# Autodesk Inventor assembly: Leg_joint_roll_yaw
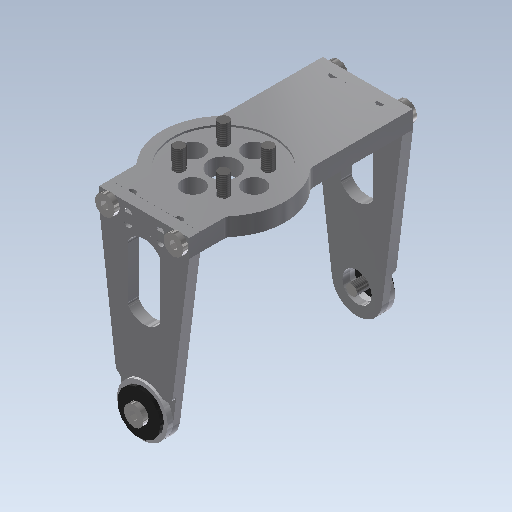
[picture p0: Inventor's stored thumbnail of the model, 512x512]
Saved by Autodesk Inventor 2020 (Build 240168000, 168)
## iProperties
Created: 2016-05-01
Part Number: Leg_joint_roll_yaw
Document SubType Name: Assembly
Designer: hiroaki
Mass: 101.489 g
Surface Area: 218.083 cm^2
Volume: 17.9148 cm^3
Density: 5.6651 g/cm^3
Author: hiroaki
## Documents named in this file (7)
- C:\Users\Masato\Documents\Inventor\CIT Brains_Inventor\OpenPlatform_ver3_0\LowerBody\Leg_joit\Leg_joint_roll_yaw.iam
- C:\Users\Masato\Documents\Inventor\CIT Brains_Inventor\OpenPlatform_ver3_0\Ready_Made\UUW-0312-10BH.ipt
- C:\Users\Masato\Documents\Inventor\CIT Brains_Inventor\OpenPlatform_ver3_0\LowerBody\Leg_joit\Leg_joint_yaw_frame.ipt
- C:\Users\Masato\Documents\Inventor\CIT Brains_Inventor\OpenPlatform_ver3_0\Ready_Made\Screw\M3-10.ipt
- C:\Users\Masato\Documents\Inventor\CIT Brains_Inventor\OpenPlatform_ver3_0\Ready_Made\Screw\M3-6.ipt
- C:\Users\Masato\Documents\Inventor\CIT Brains_Inventor\OpenPlatform_ver3_0\Ready_Made\TT-0814-15.ipt
- C:\Users\Masato\Documents\Inventor\CIT Brains_Inventor\OpenPlatform_ver3_0\LowerBody\Leg_joit\Leg_joint_slider_frame.ipt
## Components (17 placed, 6 different names)
1. UUW-0312-10BH:3 — 挿入:63, 挿入:76
2. UUW-0312-10BH:4 — 挿入:64, 挿入:77
3. Leg_joint_yaw_frame:1 — 挿入:53, 挿入:54, 挿入:55, 挿入:56, 挿入:66, 挿入:67, 挿入:71, 挿入:72
4. M3-10:1 — 挿入:53
5. M3-10:2 — 挿入:54
6. M3-10:3 — 挿入:55
7. M3-10:4 — 挿入:56
8. M3-6:1 — 挿入:74
9. M3-6:2 — 挿入:73
10. M3-6:3 — 挿入:68
11. M3-6:4 — 挿入:69
12. TT-0814-15:1 — 挿入:64, 挿入:70
13. TT-0814-15:2 — 挿入:63, 挿入:75
14. Leg_joint_slider_frame:1 — 挿入:66, 挿入:67, 挿入:68, 挿入:69, 挿入:70
15. Leg_joint_slider_frame:2 — 挿入:71, 挿入:72, 挿入:73, 挿入:74, 挿入:75
16. M3-10:5 — 挿入:76
17. M3-6:5 — 挿入:77
## Relationships (18: Insert 18)
- 挿入:53 [Insert]: Leg_joint_yaw_frame:1 ↔ M3-10:1
- 挿入:54 [Insert]: Leg_joint_yaw_frame:1 ↔ M3-10:2
- 挿入:55 [Insert]: Leg_joint_yaw_frame:1 ↔ M3-10:3
- 挿入:56 [Insert]: Leg_joint_yaw_frame:1 ↔ M3-10:4
- 挿入:63 [Insert]: UUW-0312-10BH:3 ↔ TT-0814-15:2
- 挿入:64 [Insert]: UUW-0312-10BH:4 ↔ TT-0814-15:1
- 挿入:66 [Insert]: Leg_joint_yaw_frame:1 ↔ Leg_joint_slider_frame:1
- 挿入:67 [Insert]: Leg_joint_yaw_frame:1 ↔ Leg_joint_slider_frame:1
- 挿入:68 [Insert]: M3-6:3 ↔ Leg_joint_slider_frame:1
- 挿入:69 [Insert]: M3-6:4 ↔ Leg_joint_slider_frame:1
- 挿入:70 [Insert]: TT-0814-15:1 ↔ Leg_joint_slider_frame:1
- 挿入:71 [Insert]: Leg_joint_yaw_frame:1 ↔ Leg_joint_slider_frame:2
- 挿入:72 [Insert]: Leg_joint_yaw_frame:1 ↔ Leg_joint_slider_frame:2
- 挿入:73 [Insert]: M3-6:2 ↔ Leg_joint_slider_frame:2
- 挿入:74 [Insert]: M3-6:1 ↔ Leg_joint_slider_frame:2
- 挿入:75 [Insert]: TT-0814-15:2 ↔ Leg_joint_slider_frame:2
- 挿入:76 [Insert]: UUW-0312-10BH:3 ↔ M3-10:5
- 挿入:77 [Insert]: UUW-0312-10BH:4 ↔ M3-6:5
